# Autodesk Inventor assembly: POKRYWA_TYLNA
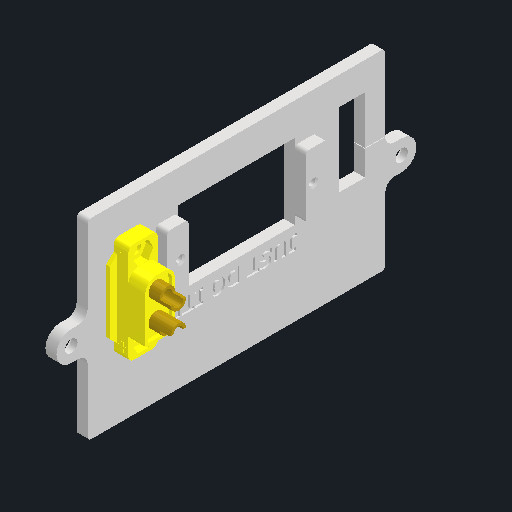
[picture p0: Inventor's stored thumbnail of the model, 512x512]
Saved by Autodesk Inventor 2023.4 (Build 274418000, 418)
## iProperties
Created: 2024-10-18
Part Number: POKRYWA_TYLNA
Document SubType Name: Assembly
Designer: komputer
Author: komputer
## Documents named in this file (3)
- E:\PROJECTS_REPOS\Robal-2.0\mechanics\POKRYWA_TYLNA.iam
- E:\PROJECTS_REPOS\Robal-2.0\mechanics\pokrywa_tyl.ipt
- E:\PROJECTS_REPOS\Robal-2.0\mechanics\XT60E-M\XT60E-M.ipt
## Components (2 placed, 2 different names)
1. pokrywa_tyl:1 — Mate:1, Flush:1, Mate:2
2. XT60E-M:1 — Mate:1, Flush:1, Mate:2
## Relationships (3: Mate 2, Flush 1)
- Mate:1: pokrywa_tyl:1 ↔ XT60E-M:1
- Flush:1 (7 mm): pokrywa_tyl:1 ↔ XT60E-M:1
- Mate:2: pokrywa_tyl:1 ↔ XT60E-M:1
